# Autodesk Inventor assembly: POM_T5_30
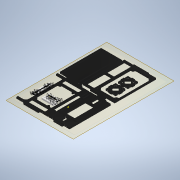
[picture p0: Inventor's stored thumbnail of the model, 180x180]
Saved by Autodesk Inventor 2020 (Build 240168000, 168)
## iProperties
Created: 2021-08-27
Part Number: POM_T5_30
Document SubType Name: Assembly
Designer: Masato
Author: Masato
## Documents named in this file (10)
- C:\Inventor\SUSTAINA-OP\Cam\POM_T5_30.iam
- C:\Inventor\SUSTAINA-OP\Cam\DisposableBoard.ipt
- C:\Inventor\SUSTAINA-OP\UpperBody\Arm\UpperArm_diagonal.ipt
- C:\Inventor\SUSTAINA-OP\UpperBody\Cockpit\Cockpit_carrier_board_frame.ipt
- C:\Inventor\SUSTAINA-OP\UpperBody\Cockpit\Cockpit_front_frame.ipt
- C:\Inventor\SUSTAINA-OP\UpperBody\Cockpit\Cockpit_circuit_board_frame.ipt
- C:\Inventor\SUSTAINA-OP\UpperBody\Cockpit\Cockpit_back_frame.ipt
- C:\Inventor\SUSTAINA-OP\Jig\UpperArm_diagonal_Jig.ipt
- C:\Inventor\SUSTAINA-OP\Jig\ForeArm_diagonal_Jig_1.ipt
- C:\Inventor\SUSTAINA-OP\Jig\ForeArm_diagonal_Jig_2.ipt
## Components (10 placed, 9 different names)
1. DisposableBoard:1 — メイト:2, メイト:1, フラッシュ:1, フラッシュ:2, メイト:39, メイト:40, メイト:41, メイト:42, フラッシュ:3, フラッシュ:4, メイト:44, メイト:50, メイト:51, メイト:52
2. Cockpit_carrier_board_frame:1 — メイト:40, フラッシュ:3, フラッシュ:4, フラッシュ:5, メイト:43, メイト:45, フラッシュ:6, メイト:53, メイト:55, メイト:56
3. Cockpit_front_frame:1 — メイト:41, フラッシュ:5, メイト:43, メイト:48
4. Cockpit_circuit_board_frame:1 — メイト:42, メイト:46, メイト:47, メイト:48, メイト:49
5. Cockpit_back_frame:1 — メイト:44, メイト:45, フラッシュ:6, メイト:47
6. UpperArm_diagonal_Jig:1 — メイト:50, フラッシュ:7, フラッシュ:8, メイト:54, メイト:55, メイト:56
7. ForeArm_diagonal_Jig_1:1 — メイト:51, メイト:53, フラッシュ:7
8. ForeArm_diagonal_Jig_2:1 — メイト:52, フラッシュ:8, メイト:54
9. UpperArm_diagonal:1 — メイト:39, メイト:46, メイト:49
10. UpperArm_diagonal:2
## Component patterns: (2 elements, first: UpperArm_diagonal:1)
## Relationships (28: Mate 20, Flush 8)
- メイト:2 [Mate]: DisposableBoard:1
- メイト:1 [Mate]: DisposableBoard:1
- フラッシュ:1 [Flush]: DisposableBoard:1
- フラッシュ:2 [Flush]: DisposableBoard:1
- メイト:39 [Mate]: DisposableBoard:1 ↔ UpperArm_diagonal:1
- メイト:40 [Mate]: DisposableBoard:1 ↔ Cockpit_carrier_board_frame:1
- メイト:41 [Mate]: DisposableBoard:1 ↔ Cockpit_front_frame:1
- メイト:42 [Mate]: DisposableBoard:1 ↔ Cockpit_circuit_board_frame:1
- フラッシュ:3 [Flush] (2 mm): DisposableBoard:1 ↔ Cockpit_carrier_board_frame:1
- フラッシュ:4 [Flush] (2 mm): DisposableBoard:1 ↔ Cockpit_carrier_board_frame:1
- フラッシュ:5 [Flush]: Cockpit_carrier_board_frame:1 ↔ Cockpit_front_frame:1
- メイト:43 [Mate] (2.5 mm): Cockpit_carrier_board_frame:1 ↔ Cockpit_front_frame:1
- メイト:44 [Mate]: DisposableBoard:1 ↔ Cockpit_back_frame:1
- メイト:45 [Mate] (2.5 mm): Cockpit_carrier_board_frame:1 ↔ Cockpit_back_frame:1
- フラッシュ:6 [Flush]: Cockpit_carrier_board_frame:1 ↔ Cockpit_back_frame:1
- メイト:46 [Mate] (10 mm): Cockpit_circuit_board_frame:1 ↔ UpperArm_diagonal:1
- メイト:47 [Mate] (2.5 mm): Cockpit_circuit_board_frame:1 ↔ Cockpit_back_frame:1
- メイト:48 [Mate] (2.5 mm): Cockpit_front_frame:1 ↔ Cockpit_circuit_board_frame:1
- メイト:49 [Mate] (13 mm): Cockpit_circuit_board_frame:1 ↔ UpperArm_diagonal:1
- メイト:50 [Mate]: DisposableBoard:1 ↔ UpperArm_diagonal_Jig:1
- メイト:51 [Mate]: DisposableBoard:1 ↔ ForeArm_diagonal_Jig_1:1
- メイト:52 [Mate]: DisposableBoard:1 ↔ ForeArm_diagonal_Jig_2:1
- メイト:53 [Mate] (2.5 mm): Cockpit_carrier_board_frame:1 ↔ ForeArm_diagonal_Jig_1:1
- フラッシュ:7 [Flush]: UpperArm_diagonal_Jig:1 ↔ ForeArm_diagonal_Jig_1:1
- フラッシュ:8 [Flush]: UpperArm_diagonal_Jig:1 ↔ ForeArm_diagonal_Jig_2:1
- メイト:54 [Mate] (2.5 mm): UpperArm_diagonal_Jig:1 ↔ ForeArm_diagonal_Jig_2:1
- メイト:55 [Mate] (13 mm): Cockpit_carrier_board_frame:1 ↔ UpperArm_diagonal_Jig:1
- メイト:56 [Mate] (13 mm): Cockpit_carrier_board_frame:1 ↔ UpperArm_diagonal_Jig:1
